# Autodesk Inventor assembly: Omni Alpha 1
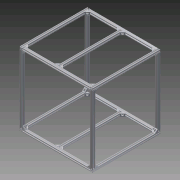
[picture p0: Inventor's stored thumbnail of the model, 180x180]
Saved by Autodesk Inventor 2015 (Build 190159000, 159)
## iProperties
Created: 2015-08-10
Part Number: Omni Alpha 1
Document SubType Name: Assembly
Designer: Solomon
Author: Solomon
## Documents named in this file (4)
- C:\Users\Solomon\Documents\Inventor\Omni 1\Omni Alpha 1.iam
- C:\Users\Solomon\Documents\Inventor\Omni 1\V Slot Part Files\Extrusions\vslot 20 x 20 v2.ipt
- C:\Users\Solomon\Documents\Inventor\Omni 1\vslot 20 x 20_40mm short.ipt
- C:\Users\Solomon\Documents\Inventor\Omni 1\V Slot Part Files\Brackets and Joining Plates\90 Degree Corner Connector.ipt
## Components (46 placed, 3 different names)
1. vslot 20 x 20 v2:1 — Angle:1, Mate:1, Flush:1, Flush:3, Mate:3, Flush:5, Flush:12, Mate:53, Mate:58, Flush:48, Mate:71, Mate:75
2. vslot 20 x 20 v2:2 — Angle:1, Mate:1, Flush:1, Angle:2, Mate:2, Flush:2, Flush:11, Flush:12, Mate:19, Mate:44, Flush:40, Angle:8, Mate:52, Flush:45, Mate:78, Flush:58
3. vslot 20 x 20 v2:3 — Angle:2, Mate:2, Flush:2, Flush:4, Mate:4, Flush:6, Flush:11, Mate:14, Flush:25, Angle:5, Mate:37, Flush:36, Mate:38, Flush:37, Mate:40, Flush:38, Mate:45, Mate:70, Flush:54, Mate:77
4. vslot 20 x 20 v2:4 — Flush:3, Mate:3, Flush:5, Mate:7, Flush:13, Flush:14, Mate:11, Flush:22, Flush:23, Mate:13, Mate:17, Flush:26, Mate:47, Flush:42, Angle:7, Mate:49, Mate:59
5. vslot 20 x 20 v2:5 — Mate:5, Flush:7, Flush:8, Mate:6, Flush:9, Flush:10, Mate:54, Flush:46, Mate:57, Flush:47, Mate:72, Flush:55, Mate:76, Flush:57
6. vslot 20 x 20 v2:6 — Flush:4, Mate:4, Flush:6, Mate:5, Flush:7, Flush:8, Flush:19, Mate:10, Flush:20, Flush:21, Mate:15, Mate:28, Mate:39, Mate:55, Angle:11, Mate:61, Flush:49
7. vslot 20 x 20 v2:7 — Mate:6, Flush:9, Flush:10, Mate:8, Flush:15, Flush:16, Mate:9, Flush:17, Flush:18, Mate:31, Mate:34, Flush:35, Mate:51, Angle:9, Mate:56
8. vslot 20 x 20 v2:8 — Mate:7, Flush:13, Flush:14, Angle:3, Flush:24, Mate:32, Flush:34, Mate:35, Mate:43, Mate:46, Flush:41, Mate:73, Mate:74, Flush:56
9. vslot 20 x 20 v2:9 — Mate:11, Flush:22, Flush:23, Mate:48, Flush:43, Angle:15, Mate:67, Mate:69, Mate:79
10. vslot 20 x 20 v2:10 — Mate:10, Flush:20, Flush:21, Flush:27, Mate:18, Mate:22, Flush:29, Mate:24, Flush:30, Flush:32, Mate:29, Angle:12, Mate:63, Mate:68, Flush:53
11. vslot 20 x 20 v2:11 — Mate:9, Flush:17, Flush:18, Flush:19, Mate:50, Flush:44, Angle:10, Mate:60, Angle:13, Mate:62, Flush:50, Mate:65
12. vslot 20 x 20 v2:12 — Mate:8, Flush:15, Flush:16, Mate:12, Mate:16, Mate:20, Mate:27, Flush:31, Mate:30, Flush:33, Mate:64, Flush:51, Mate:66, Flush:52
13. vslot 20 x 20_40mm short:1 — Angle:3, Mate:12, Flush:24, Mate:13, Mate:21, Flush:28, Mate:26, Mate:33, Mate:42, Flush:39, Angle:14
14. vslot 20 x 20_40mm short:2 — Mate:14, Flush:25, Mate:15, Mate:23, Angle:4, Mate:25, Mate:36, Angle:6, Mate:41
15. 90 Degree Corner Connector:1 — Mate:16, Mate:17, Flush:26
16. 90 Degree Corner Connector:2 — Flush:27, Mate:18, Mate:19
17. 90 Degree Corner Connector:3 — Mate:20, Mate:21, Flush:28
18. 90 Degree Corner Connector:4 — Mate:22, Mate:23, Flush:29
19. 90 Degree Corner Connector:5 — Mate:24, Angle:4, Flush:30, Mate:25
20. 90 Degree Corner Connector:6 — Mate:26, Mate:27, Flush:31
21. 90 Degree Corner Connector:7 — Mate:28, Flush:32, Mate:29
22. 90 Degree Corner Connector:8 — Mate:30, Flush:33, Mate:31
23. 90 Degree Corner Connector:10 — Angle:5, Mate:32, Mate:33, Flush:34
24. 90 Degree Corner Connector:11 — Mate:34, Flush:35, Mate:35
25. 90 Degree Corner Connector:12 — Mate:36, Mate:37, Flush:36
26. 90 Degree Corner Connector:13 — Mate:38, Mate:39, Flush:37
27. 90 Degree Corner Connector:14 — Angle:6, Mate:40, Mate:41, Flush:38
28. 90 Degree Corner Connector:15 — Mate:42, Mate:43, Flush:39
29. 90 Degree Corner Connector:16 — Mate:44, Mate:45, Flush:40
30. 90 Degree Corner Connector:17 — Mate:46, Mate:47, Flush:41, Flush:42
31. 90 Degree Corner Connector:18 — Angle:7, Mate:48, Flush:43, Mate:49
32. 90 Degree Corner Connector:19 — Mate:50, Mate:51, Flush:44
33. 90 Degree Corner Connector:20 — Angle:8, Mate:52, Mate:53, Flush:45
34. 90 Degree Corner Connector:21 — Mate:54, Mate:55, Flush:46
35. 90 Degree Corner Connector:22 — Angle:9, Mate:56, Mate:57, Flush:47
36. 90 Degree Corner Connector:23 — Mate:58, Mate:59, Flush:48
37. 90 Degree Corner Connector:24 — Angle:10, Angle:11, Mate:60, Mate:61, Flush:49
38. 90 Degree Corner Connector:25 — Angle:12, Mate:68, Mate:69, Flush:53
39. 90 Degree Corner Connector:26 — Angle:13, Mate:62, Mate:63, Flush:50
40. 90 Degree Corner Connector:27 — Angle:14, Mate:64, Mate:65, Flush:51
41. 90 Degree Corner Connector:28 — Angle:15, Mate:66, Mate:67, Flush:52
42. 90 Degree Corner Connector:29 — Mate:70, Mate:71, Flush:54
43. 90 Degree Corner Connector:30 — Mate:76, Mate:77, Flush:57
44. 90 Degree Corner Connector:31 — Mate:72, Mate:73, Flush:55
45. 90 Degree Corner Connector:32 — Mate:74, Mate:75, Flush:56
46. 90 Degree Corner Connector:33 — Mate:78, Mate:79, Flush:58
## Relationships (152: Mate 79, Flush 58, Angle 15)
- Angle:1 (90 deg): vslot 20 x 20 v2:1 ↔ vslot 20 x 20 v2:2
- Mate:1 (6.1 mm): vslot 20 x 20 v2:1 ↔ vslot 20 x 20 v2:2
- Flush:1: vslot 20 x 20 v2:1 ↔ vslot 20 x 20 v2:2
- Angle:2 (0 deg): vslot 20 x 20 v2:2 ↔ vslot 20 x 20 v2:3
- Mate:2 (6.1 mm): vslot 20 x 20 v2:2 ↔ vslot 20 x 20 v2:3
- Flush:2: vslot 20 x 20 v2:2 ↔ vslot 20 x 20 v2:3
- Flush:3: vslot 20 x 20 v2:1 ↔ vslot 20 x 20 v2:4
- Mate:3 (6.1 mm): vslot 20 x 20 v2:1 ↔ vslot 20 x 20 v2:4
- Flush:4: vslot 20 x 20 v2:3 ↔ vslot 20 x 20 v2:6
- Mate:4 (6.1 mm): vslot 20 x 20 v2:3 ↔ vslot 20 x 20 v2:6
- Flush:5: vslot 20 x 20 v2:1 ↔ vslot 20 x 20 v2:4
- Flush:6: vslot 20 x 20 v2:3 ↔ vslot 20 x 20 v2:6
- Mate:5 (6.1 mm): vslot 20 x 20 v2:5 ↔ vslot 20 x 20 v2:6
- Flush:7: vslot 20 x 20 v2:5 ↔ vslot 20 x 20 v2:6
- Flush:8: vslot 20 x 20 v2:5 ↔ vslot 20 x 20 v2:6
- Mate:6 (6.1 mm): vslot 20 x 20 v2:5 ↔ vslot 20 x 20 v2:7
- Flush:9: vslot 20 x 20 v2:5 ↔ vslot 20 x 20 v2:7
- Flush:10: vslot 20 x 20 v2:5 ↔ vslot 20 x 20 v2:7
- Flush:11: vslot 20 x 20 v2:2 ↔ vslot 20 x 20 v2:3
- Flush:12: vslot 20 x 20 v2:1 ↔ vslot 20 x 20 v2:2
- Mate:7 (6.1 mm): vslot 20 x 20 v2:4 ↔ vslot 20 x 20 v2:8
- Flush:13: vslot 20 x 20 v2:4 ↔ vslot 20 x 20 v2:8
- Flush:14: vslot 20 x 20 v2:4 ↔ vslot 20 x 20 v2:8
- Mate:8 (6.1 mm): vslot 20 x 20 v2:7 ↔ vslot 20 x 20 v2:12
- Flush:15: vslot 20 x 20 v2:7 ↔ vslot 20 x 20 v2:12
- Flush:16: vslot 20 x 20 v2:7 ↔ vslot 20 x 20 v2:12
- Mate:9 (6.1 mm): vslot 20 x 20 v2:7 ↔ vslot 20 x 20 v2:11
- Flush:17: vslot 20 x 20 v2:7 ↔ vslot 20 x 20 v2:11
- Flush:18: vslot 20 x 20 v2:7 ↔ vslot 20 x 20 v2:11
- Flush:19: vslot 20 x 20 v2:6 ↔ vslot 20 x 20 v2:11
- Mate:10 (6.1 mm): vslot 20 x 20 v2:6 ↔ vslot 20 x 20 v2:10
- Flush:20: vslot 20 x 20 v2:6 ↔ vslot 20 x 20 v2:10
- Flush:21: vslot 20 x 20 v2:6 ↔ vslot 20 x 20 v2:10
- Mate:11 (6.1 mm): vslot 20 x 20 v2:4 ↔ vslot 20 x 20 v2:9
- Flush:22: vslot 20 x 20 v2:4 ↔ vslot 20 x 20 v2:9
- Flush:23: vslot 20 x 20 v2:4 ↔ vslot 20 x 20 v2:9
- Angle:3 (0 deg): vslot 20 x 20 v2:8 ↔ vslot 20 x 20_40mm short:1
- Mate:12 (6.1 mm): vslot 20 x 20 v2:12 ↔ vslot 20 x 20_40mm short:1
- Flush:24: vslot 20 x 20 v2:8 ↔ vslot 20 x 20_40mm short:1
- Mate:13 (240 mm): vslot 20 x 20 v2:4 ↔ vslot 20 x 20_40mm short:1
- Mate:14 (6.1 mm): vslot 20 x 20 v2:3 ↔ vslot 20 x 20_40mm short:2
- Flush:25: vslot 20 x 20 v2:3 ↔ vslot 20 x 20_40mm short:2
- Mate:15 (240 mm): vslot 20 x 20 v2:6 ↔ vslot 20 x 20_40mm short:2
- Mate:16 (6.1 mm): vslot 20 x 20 v2:12 ↔ 90 Degree Corner Connector:1
- Mate:17: vslot 20 x 20 v2:4 ↔ 90 Degree Corner Connector:1
- Flush:26: vslot 20 x 20 v2:4 ↔ 90 Degree Corner Connector:1
- Flush:27: vslot 20 x 20 v2:10 ↔ 90 Degree Corner Connector:2
- Mate:18: vslot 20 x 20 v2:10 ↔ 90 Degree Corner Connector:2
- Mate:19: vslot 20 x 20 v2:2 ↔ 90 Degree Corner Connector:2
- Mate:20: vslot 20 x 20 v2:12 ↔ 90 Degree Corner Connector:3
- Mate:21: vslot 20 x 20_40mm short:1 ↔ 90 Degree Corner Connector:3
- Flush:28: vslot 20 x 20_40mm short:1 ↔ 90 Degree Corner Connector:3
- Mate:22: vslot 20 x 20 v2:10 ↔ 90 Degree Corner Connector:4
- Mate:23: vslot 20 x 20_40mm short:2 ↔ 90 Degree Corner Connector:4
- Flush:29: vslot 20 x 20 v2:10 ↔ 90 Degree Corner Connector:4
- Mate:24: vslot 20 x 20 v2:10 ↔ 90 Degree Corner Connector:5
- Angle:4 (270 deg): vslot 20 x 20_40mm short:2 ↔ 90 Degree Corner Connector:5
- Flush:30: vslot 20 x 20 v2:10 ↔ 90 Degree Corner Connector:5
- Mate:25: vslot 20 x 20_40mm short:2 ↔ 90 Degree Corner Connector:5
- Mate:26: vslot 20 x 20_40mm short:1 ↔ 90 Degree Corner Connector:6
- Mate:27: vslot 20 x 20 v2:12 ↔ 90 Degree Corner Connector:6
- Flush:31: vslot 20 x 20 v2:12 ↔ 90 Degree Corner Connector:6
- Mate:28: vslot 20 x 20 v2:6 ↔ 90 Degree Corner Connector:7
- Flush:32: vslot 20 x 20 v2:10 ↔ 90 Degree Corner Connector:7
- Mate:29: vslot 20 x 20 v2:10 ↔ 90 Degree Corner Connector:7
- Mate:30: vslot 20 x 20 v2:12 ↔ 90 Degree Corner Connector:8
- Flush:33: vslot 20 x 20 v2:12 ↔ 90 Degree Corner Connector:8
- Mate:31: vslot 20 x 20 v2:7 ↔ 90 Degree Corner Connector:8
- Angle:5 (0 deg): vslot 20 x 20 v2:3 ↔ 90 Degree Corner Connector:10
- Mate:32: vslot 20 x 20 v2:8 ↔ 90 Degree Corner Connector:10
- Mate:33: vslot 20 x 20_40mm short:1 ↔ 90 Degree Corner Connector:10
- Flush:34: vslot 20 x 20 v2:8 ↔ 90 Degree Corner Connector:10
- Mate:34: vslot 20 x 20 v2:7 ↔ 90 Degree Corner Connector:11
- Flush:35: vslot 20 x 20 v2:7 ↔ 90 Degree Corner Connector:11
- Mate:35: vslot 20 x 20 v2:8 ↔ 90 Degree Corner Connector:11
- Mate:36: vslot 20 x 20_40mm short:2 ↔ 90 Degree Corner Connector:12
- Mate:37: vslot 20 x 20 v2:3 ↔ 90 Degree Corner Connector:12
- Flush:36: vslot 20 x 20 v2:3 ↔ 90 Degree Corner Connector:12
- Mate:38: vslot 20 x 20 v2:3 ↔ 90 Degree Corner Connector:13
- Mate:39: vslot 20 x 20 v2:6 ↔ 90 Degree Corner Connector:13
- Flush:37: vslot 20 x 20 v2:3 ↔ 90 Degree Corner Connector:13
- Angle:6 (0 deg): vslot 20 x 20_40mm short:2 ↔ 90 Degree Corner Connector:14
- Mate:40: vslot 20 x 20 v2:3 ↔ 90 Degree Corner Connector:14
- Mate:41: vslot 20 x 20_40mm short:2 ↔ 90 Degree Corner Connector:14
- Flush:38: vslot 20 x 20 v2:3 ↔ 90 Degree Corner Connector:14
- Mate:42: vslot 20 x 20_40mm short:1 ↔ 90 Degree Corner Connector:15
- Mate:43: vslot 20 x 20 v2:8 ↔ 90 Degree Corner Connector:15
- Flush:39: vslot 20 x 20_40mm short:1 ↔ 90 Degree Corner Connector:15
- Mate:44: vslot 20 x 20 v2:2 ↔ 90 Degree Corner Connector:16
- Mate:45: vslot 20 x 20 v2:3 ↔ 90 Degree Corner Connector:16
- Flush:40: vslot 20 x 20 v2:2 ↔ 90 Degree Corner Connector:16
- Mate:46: vslot 20 x 20 v2:8 ↔ 90 Degree Corner Connector:17
- Mate:47: vslot 20 x 20 v2:4 ↔ 90 Degree Corner Connector:17
- Flush:41: vslot 20 x 20 v2:8 ↔ 90 Degree Corner Connector:17
- Flush:42: vslot 20 x 20 v2:4 ↔ 90 Degree Corner Connector:17
- Angle:7 (0 deg): vslot 20 x 20 v2:4 ↔ 90 Degree Corner Connector:18
- Mate:48: vslot 20 x 20 v2:9 ↔ 90 Degree Corner Connector:18
- Flush:43: vslot 20 x 20 v2:9 ↔ 90 Degree Corner Connector:18
- Mate:49: vslot 20 x 20 v2:4 ↔ 90 Degree Corner Connector:18
- Mate:50: vslot 20 x 20 v2:11 ↔ 90 Degree Corner Connector:19
- Mate:51: vslot 20 x 20 v2:7 ↔ 90 Degree Corner Connector:19
- Flush:44: vslot 20 x 20 v2:11 ↔ 90 Degree Corner Connector:19
- Angle:8 (0 deg): vslot 20 x 20 v2:2 ↔ 90 Degree Corner Connector:20
- Mate:52: vslot 20 x 20 v2:2 ↔ 90 Degree Corner Connector:20
- Mate:53: vslot 20 x 20 v2:1 ↔ 90 Degree Corner Connector:20
- Flush:45: vslot 20 x 20 v2:2 ↔ 90 Degree Corner Connector:20
- Mate:54: vslot 20 x 20 v2:5 ↔ 90 Degree Corner Connector:21
- Mate:55: vslot 20 x 20 v2:6 ↔ 90 Degree Corner Connector:21
- Flush:46: vslot 20 x 20 v2:5 ↔ 90 Degree Corner Connector:21
- Angle:9 (0 deg): vslot 20 x 20 v2:7 ↔ 90 Degree Corner Connector:22
- Mate:56: vslot 20 x 20 v2:7 ↔ 90 Degree Corner Connector:22
- Mate:57: vslot 20 x 20 v2:5 ↔ 90 Degree Corner Connector:22
- Flush:47: vslot 20 x 20 v2:5 ↔ 90 Degree Corner Connector:22
- Mate:58: vslot 20 x 20 v2:1 ↔ 90 Degree Corner Connector:23
- Mate:59: vslot 20 x 20 v2:4 ↔ 90 Degree Corner Connector:23
- Flush:48: vslot 20 x 20 v2:1 ↔ 90 Degree Corner Connector:23
- Angle:10 (0 deg): vslot 20 x 20 v2:11 ↔ 90 Degree Corner Connector:24
- Angle:11 (0 deg): vslot 20 x 20 v2:6 ↔ 90 Degree Corner Connector:24
- Mate:60: vslot 20 x 20 v2:11 ↔ 90 Degree Corner Connector:24
- Mate:61: vslot 20 x 20 v2:6 ↔ 90 Degree Corner Connector:24
- Flush:49: vslot 20 x 20 v2:6 ↔ 90 Degree Corner Connector:24
- Angle:12 (0 deg): vslot 20 x 20 v2:10 ↔ 90 Degree Corner Connector:25
- Angle:13 (0 deg): vslot 20 x 20 v2:11 ↔ 90 Degree Corner Connector:26
- Angle:14 (0 deg): vslot 20 x 20_40mm short:1 ↔ 90 Degree Corner Connector:27
- Angle:15 (0 deg): vslot 20 x 20 v2:9 ↔ 90 Degree Corner Connector:28
- Mate:62: vslot 20 x 20 v2:11 ↔ 90 Degree Corner Connector:26
- Mate:63: vslot 20 x 20 v2:10 ↔ 90 Degree Corner Connector:26
- Flush:50: vslot 20 x 20 v2:11 ↔ 90 Degree Corner Connector:26
- Mate:64: vslot 20 x 20 v2:12 ↔ 90 Degree Corner Connector:27
- Mate:65: vslot 20 x 20 v2:11 ↔ 90 Degree Corner Connector:27
- Flush:51: vslot 20 x 20 v2:12 ↔ 90 Degree Corner Connector:27
- Mate:66: vslot 20 x 20 v2:12 ↔ 90 Degree Corner Connector:28
- Mate:67: vslot 20 x 20 v2:9 ↔ 90 Degree Corner Connector:28
- Flush:52: vslot 20 x 20 v2:12 ↔ 90 Degree Corner Connector:28
- Mate:68: vslot 20 x 20 v2:10 ↔ 90 Degree Corner Connector:25
- Mate:69: vslot 20 x 20 v2:9 ↔ 90 Degree Corner Connector:25
- Flush:53: vslot 20 x 20 v2:10 ↔ 90 Degree Corner Connector:25
- Mate:70: vslot 20 x 20 v2:3 ↔ 90 Degree Corner Connector:29
- Mate:71: vslot 20 x 20 v2:1 ↔ 90 Degree Corner Connector:29
- Flush:54: vslot 20 x 20 v2:3 ↔ 90 Degree Corner Connector:29
- Mate:72: vslot 20 x 20 v2:5 ↔ 90 Degree Corner Connector:31
- Mate:73: vslot 20 x 20 v2:8 ↔ 90 Degree Corner Connector:31
- Flush:55: vslot 20 x 20 v2:5 ↔ 90 Degree Corner Connector:31
- Mate:74: vslot 20 x 20 v2:8 ↔ 90 Degree Corner Connector:32
- Mate:75: vslot 20 x 20 v2:1 ↔ 90 Degree Corner Connector:32
- Flush:56: vslot 20 x 20 v2:8 ↔ 90 Degree Corner Connector:32
- Mate:76: vslot 20 x 20 v2:5 ↔ 90 Degree Corner Connector:30
- Mate:77: vslot 20 x 20 v2:3 ↔ 90 Degree Corner Connector:30
- Flush:57: vslot 20 x 20 v2:5 ↔ 90 Degree Corner Connector:30
- Mate:78: vslot 20 x 20 v2:2 ↔ 90 Degree Corner Connector:33
- Mate:79: vslot 20 x 20 v2:9 ↔ 90 Degree Corner Connector:33
- Flush:58: vslot 20 x 20 v2:2 ↔ 90 Degree Corner Connector:33
